# Autodesk Inventor assembly: NK02-40-2-610
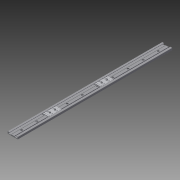
[picture p0: Inventor's stored thumbnail of the model, 180x180]
Saved by Autodesk Inventor 2013 (Build 170138000, 138)
## iProperties
Category: Plastic Bearings
Company: Autodesk, Inc.
Created: 2012-11-28
Part Number: NK02-40-2-610
Document SubType Name: Assembly
Project: FIRST
Catalog Web Link: http://www.igus.com/_Product_Files/Download/pdf/drylinn.pdf
Description: Linear guide system
Vendor: igus
Title: Linear Guide System
Author: Autodesk, Inc.
## Documents named in this file (3)
- C:\Data Folder\FIRST 2013\FIRST KOP\Parts\Plastic Bearings\PB_Bearing_NK02-40-2-610.iam
- C:\Data Folder\FIRST 2013\FIRST KOP\Parts\Plastic Bearings\NK04-40 RAIL.ipt
- C:\Data Folder\FIRST 2013\FIRST KOP\Parts\Plastic Bearings\NK04-40 CARRIAGE.ipt
## Components (3 placed, 2 different names)
1. NK04-40 RAIL:1 — Mate:1, Mate:2, Mate:3, Mate:4
2. NK04-40 CARRIAGE:1 — Mate:1, Mate:2
3. NK04-40 CARRIAGE:2 — Mate:3, Mate:4
## Relationships (4: Mate 4)
- Mate:1: NK04-40 RAIL:1 ↔ NK04-40 CARRIAGE:1
- Mate:2: NK04-40 RAIL:1 ↔ NK04-40 CARRIAGE:1
- Mate:3: NK04-40 RAIL:1 ↔ NK04-40 CARRIAGE:2
- Mate:4: NK04-40 RAIL:1 ↔ NK04-40 CARRIAGE:2
